# Autodesk Inventor assembly: The hook mechanism thing
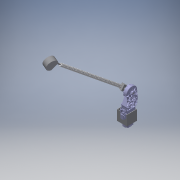
[picture p0: Inventor's stored thumbnail of the model, 180x180]
Saved by Autodesk Inventor 2016 (Build 200138000, 138)
## iProperties
Created: 2016-01-15
Part Number: The hook mechanism thing
Document SubType Name: Assembly
Designer: Administrator
Author: Administrator
## Documents named in this file (8)
- C:\Users\Administrator\Desktop\3192CAD\InitialRobotProto\parts\The hook mechanism thing.iam
- C:\Users\Administrator\Desktop\3192CAD\InitialRobotProto\parts\Churro.ipt
- C:\Users\Administrator\Desktop\3192CAD\InitialRobotProto\parts\Part2.ipt
- C:\Users\Administrator\Desktop\3192CAD\InitialRobotProto\parts\window motor.ipt
- C:\Users\Administrator\Desktop\3192CAD\InitialRobotProto\parts\really cool squares.ipt
- C:\Users\Administrator\Desktop\3192CAD\InitialRobotProto\parts\l braket w. squares.ipt
- C:\Users\Administrator\Desktop\3192CAD\InitialRobotProto\parts\bottom hook.ipt
- C:\Users\Administrator\Desktop\3192CAD\InitialRobotProto\parts\lol kill me.ipt
## Components (7 placed, 7 different names)
1. Churro:1 — Flush:2, Mate:8, Mate:9, Mate:11, Mate:12, Flush:4
2. Part2:1 — Mate:1, Mate:2, Mate:3
3. window motor:1 — Mate:1, Mate:2, Mate:3, Mate:4, Mate:5
4. really cool squares:1 — Mate:4, Mate:5, Mate:6, Mate:7, Flush:1
5. l braket w. squares:1 — Mate:6, Mate:7, Flush:1, Flush:2, Mate:8, Mate:9
6. bottom hook:1 — Mate:11, Mate:12, Flush:4, Mate:13, Flush:5, Flush:6, Flush:7
7. lol kill me:1 — Mate:13, Flush:5, Flush:6, Flush:7
## Relationships (18: Mate 12, Flush 6)
- Mate:1: Part2:1 ↔ window motor:1
- Mate:2: Part2:1 ↔ window motor:1
- Mate:3: Part2:1 ↔ window motor:1
- Mate:4: window motor:1 ↔ really cool squares:1
- Mate:5: window motor:1 ↔ really cool squares:1
- Mate:6: really cool squares:1 ↔ l braket w. squares:1
- Mate:7: really cool squares:1 ↔ l braket w. squares:1
- Flush:1: really cool squares:1 ↔ l braket w. squares:1
- Flush:2: Churro:1 ↔ l braket w. squares:1
- Mate:8: Churro:1 ↔ l braket w. squares:1
- Mate:9: Churro:1 ↔ l braket w. squares:1
- Mate:11: Churro:1 ↔ bottom hook:1
- Mate:12: Churro:1 ↔ bottom hook:1
- Flush:4 (51.308 mm): Churro:1 ↔ bottom hook:1
- Mate:13: bottom hook:1 ↔ lol kill me:1
- Flush:5: bottom hook:1 ↔ lol kill me:1
- Flush:6 (-19.5326 mm): bottom hook:1 ↔ lol kill me:1
- Flush:7 (-19.5326 mm): bottom hook:1 ↔ lol kill me:1
